# Autodesk Inventor assembly: Assembly
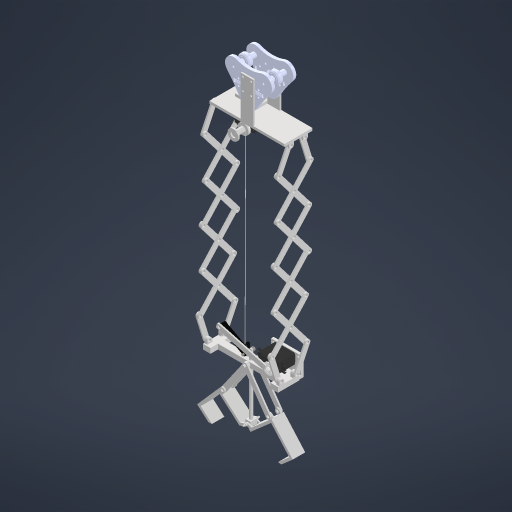
[picture p0: Inventor's stored thumbnail of the model, 512x512]
Saved by Autodesk Inventor 2023.6 (Build 276521000, 521)
## iProperties
Created: 2026-03-04
Part Number: Assembly
Document SubType Name: Assembly
Designer: user
Author: user
## Documents named in this file (19)
- D:\FP Revisi\Assembly.iam
- D:\FP Revisi\Claw New.ipt
- D:\FP Revisi\Claw New side.ipt
- D:\FP Revisi\Claw Connector 1.ipt
- D:\FP Revisi\Shaft.ipt
- D:\FP Revisi\Claw Arm.ipt
- D:\FP Revisi\Claw Connector 2.ipt
- C:\Users\user\OneDrive\Documents\FP V2 Batang Penggerak.ipt
- D:\FP Revisi\MG_996R v1.iam
- C:\Users\user\OneDrive\Documents\Inventor\Content Center Files\R2023\en-US\AS 1420\AS 1420 - 1973 - M4 x 20.ipt
- D:\FP Revisi\Lazy Tongs beam Short.ipt
- D:\FP Revisi\Lazy Tongs beam Long.ipt
- C:\Users\user\Downloads\FP_Batch 2\Sub Assembly Slider axis x.iam
- D:\FP Revisi\Mounting atas.ipt
- C:\Users\user\OneDrive\Documents\fp v2 servo Mounting.ipt
- D:\FP Revisi\MG_996R.iam
- D:\FP Revisi\Pulley Mechanism.ipt
- D:\FP Revisi\Hook.ipt
- D:\FP Revisi\Ropes.ipt
## Components (47 placed, 18 different names)
1. Claw New:1 — Mate:1, Mate:2, Mate:7, Mate:8, Mate:9, Mate:10
2. Claw New side:1 — Mate:1, Mate:2, Mate:3, Mate:4, Mate:11, Mate:12, Mate:13, Mate:14
3. Claw Connector 1:1 — Mate:3, Mate:4, Mate:5, Mate:6
4. Shaft:1 — Mate:5, Mate:6, Mate:18, Mate:20, Mate:26, Mate:35, Mate:36
5. Claw Arm:1 — Mate:11, Mate:12, Mate:15, Mate:19
6. Claw Arm:2 — Mate:7, Mate:8, Mate:15, Mate:16
7. Claw Arm:3 — Mate:9, Mate:10, Mate:17
8. Claw Arm:4 — Mate:13, Mate:14, Mate:16, Mate:17
9. Claw Connector 2:1 — Mate:18, Mate:19, Flush:1, Mate:37, Mate:38, Mate:47, Mate:48, Mate:86, Mate:87, Mate:88, Mate:89, Flush:2, Flush:3, Mate:110, Flush:4, Mate:128, Mate:129
10. FP V2 Batang Penggerak:1 — Mate:20, Mate:23, Mate:24, Mate:25, Mate:34
11. MG_996R v1:1 [sub-assembly] — Flush:1, Mate:23, Mate:24, Mate:27, Mate:32, Flush:3, Mate:111, Mate:112, Mate:113, Mate:114, Mate:115
12. FP V2 Batang Penggerak:2 — Mate:25, Mate:26, Mate:27, Mate:30, Mate:31, Mate:33
13. FP V2 Batang Penggerak:3 — Mate:28, Mate:29, Mate:31, Mate:33
14. FP V2 Batang Penggerak:4 — Mate:28, Mate:29, Mate:30, Mate:32, Mate:34
15. AS 1420 - Metric M4 x 20:1 — Mate:35, Mate:36
16. Lazy Tongs beam Short:4 — Mate:37, Mate:38, Mate:45, Mate:46
17. Lazy Tongs beam Long:1 — Mate:45, Mate:46, Mate:51, Mate:52, Mate:58
18. Lazy Tongs beam Long:2 — Mate:49, Mate:50, Mate:51, Mate:54, Mate:55
19. Lazy Tongs beam Long:3 — Mate:60, Mate:61, Mate:62, Mate:63, Mate:66
20. Lazy Tongs beam Long:4 — Mate:63, Mate:66, Mate:91, Mate:96, Mate:97
21. Lazy Tongs beam Long:5 — Mate:57, Mate:59, Mate:62, Mate:64, Mate:65
22. Lazy Tongs beam Long:6 — Mate:52, Mate:56, Mate:57, Mate:58, Mate:59
23. Lazy Tongs beam Long:7 — Mate:64, Mate:65, Mate:91, Mate:94, Mate:95
24. Lazy Tongs beam Long:8 — Mate:54, Mate:55, Mate:56, Mate:60, Mate:61
25. Lazy Tongs beam Short:5 — Mate:47, Mate:48, Mate:49, Mate:50
26. Lazy Tongs beam Short:6 — Mate:86, Mate:89
27. Lazy Tongs beam Long:9
28. Lazy Tongs beam Long:10
29. Lazy Tongs beam Long:11
30. Lazy Tongs beam Long:12 — Mate:90, Mate:100, Mate:103
31. Lazy Tongs beam Long:13
32. Lazy Tongs beam Long:14
33. Lazy Tongs beam Long:15 — Mate:90, Mate:101, Mate:102
34. Lazy Tongs beam Long:16
35. Lazy Tongs beam Short:7 — Mate:87, Mate:88
36. Mounting atas:1 — Flush:2, Mate:92, Mate:93, Mate:98, Mate:99, Mate:105, Mate:106, Mate:107, Mate:108, Mate:109, Mate:117, Mate:130
37. Lazy Tongs beam Short:9 — Mate:92, Mate:94, Mate:95
38. Lazy Tongs beam Short:10 — Mate:93, Mate:96, Mate:97
39. Lazy Tongs beam Short:11 — Mate:99, Mate:100, Mate:103
40. Lazy Tongs beam Short:12 — Mate:98, Mate:101, Mate:102
41. Sub Assembly Slider axis x:1 [sub-assembly] — Mate:105, Mate:106, Mate:107, Mate:108, Mate:109
42. fp v2 servo Mounting:1 — Mate:110, Mate:111, Mate:112, Mate:113, Mate:114, Mate:115
43. MG_996R:1 [sub-assembly] — Mate:118, Mate:119, Mate:120, Mate:121, Mate:122, Mate:123, Mate:124, Mate:125, Mate:126, Mate:127
44. fp v2 servo Mounting:2 — Mate:117, Mate:118, Mate:119, Mate:120, Mate:121, Mate:122, Mate:130
45. Pulley Mechanism:1 — Mate:123, Mate:124, Mate:125, Mate:126, Mate:127, Flush:4, Flush:5
46. Hook:1 — Mate:128, Mate:129, Flush:6, Flush:9
47. Ropes:1 — Flush:7, Flush:8, Flush:9
## Relationships (128: Mate 119, Flush 9)
- Mate:1: Claw New:1 ↔ Claw New side:1
- Mate:2: Claw New:1 ↔ Claw New side:1
- Mate:3: Claw New side:1 ↔ Claw Connector 1:1
- Mate:4: Claw New side:1 ↔ Claw Connector 1:1
- Mate:5: Claw Connector 1:1 ↔ Shaft:1
- Mate:6: Claw Connector 1:1 ↔ Shaft:1
- Mate:7: Claw New:1 ↔ Claw Arm:2
- Mate:8: Claw New:1 ↔ Claw Arm:2
- Mate:9: Claw New:1 ↔ Claw Arm:3
- Mate:10: Claw New:1 ↔ Claw Arm:3
- Mate:11: Claw New side:1 ↔ Claw Arm:1
- Mate:12: Claw New side:1 ↔ Claw Arm:1
- Mate:13: Claw New side:1 ↔ Claw Arm:4
- Mate:14: Claw New side:1 ↔ Claw Arm:4
- Mate:15: Claw Arm:1 ↔ Claw Arm:2
- Mate:16: Claw Arm:2 ↔ Claw Arm:4
- Mate:17: Claw Arm:3 ↔ Claw Arm:4
- Mate:18: Shaft:1 ↔ Claw Connector 2:1
- Mate:19: Claw Arm:1 ↔ Claw Connector 2:1
- Mate:20: Shaft:1 ↔ FP V2 Batang Penggerak:1
- Flush:1: Claw Connector 2:1 ↔ MG_996R v1:1
- Mate:23: FP V2 Batang Penggerak:1 ↔ MG_996R v1:1
- Mate:24: FP V2 Batang Penggerak:1 ↔ MG_996R v1:1
- Mate:25: FP V2 Batang Penggerak:1 ↔ FP V2 Batang Penggerak:2
- Mate:26: Shaft:1 ↔ FP V2 Batang Penggerak:2
- Mate:27: MG_996R v1:1 ↔ FP V2 Batang Penggerak:2
- Mate:28: FP V2 Batang Penggerak:3 ↔ FP V2 Batang Penggerak:4
- Mate:29: FP V2 Batang Penggerak:3 ↔ FP V2 Batang Penggerak:4
- Mate:30: FP V2 Batang Penggerak:2 ↔ FP V2 Batang Penggerak:4
- Mate:31: FP V2 Batang Penggerak:2 ↔ FP V2 Batang Penggerak:3
- Mate:32: MG_996R v1:1 ↔ FP V2 Batang Penggerak:4
- Mate:33: FP V2 Batang Penggerak:2 ↔ FP V2 Batang Penggerak:3
- Mate:34: FP V2 Batang Penggerak:1 ↔ FP V2 Batang Penggerak:4
- Mate:35: Shaft:1 ↔ AS 1420 - Metric M4 x 20:1
- Mate:36: Shaft:1 ↔ AS 1420 - Metric M4 x 20:1
- Mate:37: Claw Connector 2:1 ↔ Lazy Tongs beam Short:4
- Mate:38: Claw Connector 2:1 ↔ Lazy Tongs beam Short:4
- Mate:45: Lazy Tongs beam Short:4 ↔ Lazy Tongs beam Long:1
- Mate:46: Lazy Tongs beam Short:4 ↔ Lazy Tongs beam Long:1
- Mate:47: Claw Connector 2:1 ↔ Lazy Tongs beam Short:5
- Mate:48: Claw Connector 2:1 ↔ Lazy Tongs beam Short:5
- Mate:49: Lazy Tongs beam Long:2 ↔ Lazy Tongs beam Short:5
- Mate:50: Lazy Tongs beam Long:2 ↔ Lazy Tongs beam Short:5
- Mate:51: Lazy Tongs beam Long:1 ↔ Lazy Tongs beam Long:2
- Mate:52: Lazy Tongs beam Long:1 ↔ Lazy Tongs beam Long:6
- Mate:54: Lazy Tongs beam Long:2 ↔ Lazy Tongs beam Long:8
- Mate:55: Lazy Tongs beam Long:2 ↔ Lazy Tongs beam Long:8
- Mate:56: Lazy Tongs beam Long:6 ↔ Lazy Tongs beam Long:8
- Mate:57: Lazy Tongs beam Long:5 ↔ Lazy Tongs beam Long:6
- Mate:58: Lazy Tongs beam Long:1 ↔ Lazy Tongs beam Long:6
- Mate:59: Lazy Tongs beam Long:5 ↔ Lazy Tongs beam Long:6
- Mate:60: Lazy Tongs beam Long:3 ↔ Lazy Tongs beam Long:8
- Mate:61: Lazy Tongs beam Long:3 ↔ Lazy Tongs beam Long:8
- Mate:62: Lazy Tongs beam Long:3 ↔ Lazy Tongs beam Long:5
- Mate:63: Lazy Tongs beam Long:3 ↔ Lazy Tongs beam Long:4
- Mate:64: Lazy Tongs beam Long:5 ↔ Lazy Tongs beam Long:7
- Mate:65: Lazy Tongs beam Long:5 ↔ Lazy Tongs beam Long:7
- Mate:66: Lazy Tongs beam Long:3 ↔ Lazy Tongs beam Long:4
- [Mate]: Lazy Tongs beam Short:6 ↔ Lazy Tongs beam Long:9
- [Mate]: Lazy Tongs beam Short:6 ↔ Lazy Tongs beam Long:9
- [Mate]: Lazy Tongs beam Long:10 ↔ Lazy Tongs beam Short:7
- [Mate]: Lazy Tongs beam Long:10 ↔ Lazy Tongs beam Short:7
- [Mate]: Lazy Tongs beam Long:9 ↔ Lazy Tongs beam Long:10
- [Mate]: Lazy Tongs beam Long:9 ↔ Lazy Tongs beam Long:14
- [Mate]: Lazy Tongs beam Long:10 ↔ Lazy Tongs beam Long:16
- [Mate]: Lazy Tongs beam Long:10 ↔ Lazy Tongs beam Long:16
- [Mate]: Lazy Tongs beam Long:14 ↔ Lazy Tongs beam Long:16
- [Mate]: Lazy Tongs beam Long:13 ↔ Lazy Tongs beam Long:14
- [Mate]: Lazy Tongs beam Long:9 ↔ Lazy Tongs beam Long:14
- [Mate]: Lazy Tongs beam Long:13 ↔ Lazy Tongs beam Long:14
- [Mate]: Lazy Tongs beam Long:11 ↔ Lazy Tongs beam Long:16
- [Mate]: Lazy Tongs beam Long:11 ↔ Lazy Tongs beam Long:16
- [Mate]: Lazy Tongs beam Long:11 ↔ Lazy Tongs beam Long:13
- [Mate]: Lazy Tongs beam Long:11 ↔ Lazy Tongs beam Long:12
- [Mate]: Lazy Tongs beam Long:13 ↔ Lazy Tongs beam Long:15
- [Mate]: Lazy Tongs beam Long:13 ↔ Lazy Tongs beam Long:15
- [Mate]: Lazy Tongs beam Long:11 ↔ Lazy Tongs beam Long:12
- Mate:86: Claw Connector 2:1 ↔ Lazy Tongs beam Short:6
- Mate:87: Claw Connector 2:1 ↔ Lazy Tongs beam Short:7
- Mate:88: Claw Connector 2:1 ↔ Lazy Tongs beam Short:7
- Mate:89: Claw Connector 2:1 ↔ Lazy Tongs beam Short:6
- Mate:90: Lazy Tongs beam Long:12 ↔ Lazy Tongs beam Long:15
- Mate:91: Lazy Tongs beam Long:4 ↔ Lazy Tongs beam Long:7
- Flush:2: Claw Connector 2:1 ↔ Mounting atas:1
- Mate:92: Mounting atas:1 ↔ Lazy Tongs beam Short:9
- Mate:93: Mounting atas:1 ↔ Lazy Tongs beam Short:10
- Mate:94: Lazy Tongs beam Long:7 ↔ Lazy Tongs beam Short:9
- Mate:95: Lazy Tongs beam Long:7 ↔ Lazy Tongs beam Short:9
- Mate:96: Lazy Tongs beam Long:4 ↔ Lazy Tongs beam Short:10
- Mate:97: Lazy Tongs beam Long:4 ↔ Lazy Tongs beam Short:10
- Mate:98: Mounting atas:1 ↔ Lazy Tongs beam Short:12
- Mate:99: Mounting atas:1 ↔ Lazy Tongs beam Short:11
- Mate:100: Lazy Tongs beam Long:12 ↔ Lazy Tongs beam Short:11
- Mate:101: Lazy Tongs beam Long:15 ↔ Lazy Tongs beam Short:12
- Mate:102: Lazy Tongs beam Long:15 ↔ Lazy Tongs beam Short:12
- Mate:103: Lazy Tongs beam Long:12 ↔ Lazy Tongs beam Short:11
- Mate:105: Mounting atas:1 ↔ Sub Assembly Slider axis x:1
- Mate:106: Mounting atas:1 ↔ Sub Assembly Slider axis x:1
- Mate:107: Mounting atas:1 ↔ Sub Assembly Slider axis x:1
- Mate:108: Mounting atas:1 ↔ Sub Assembly Slider axis x:1
- Mate:109: Mounting atas:1 ↔ Sub Assembly Slider axis x:1
- Flush:3 (16.5 mm): Claw Connector 2:1 ↔ MG_996R v1:1
- Mate:110: Claw Connector 2:1 ↔ fp v2 servo Mounting:1
- Mate:111: MG_996R v1:1 ↔ fp v2 servo Mounting:1
- Mate:112: MG_996R v1:1 ↔ fp v2 servo Mounting:1
- Mate:113: MG_996R v1:1 ↔ fp v2 servo Mounting:1
- Mate:114: MG_996R v1:1 ↔ fp v2 servo Mounting:1
- Mate:115: MG_996R v1:1 ↔ fp v2 servo Mounting:1
- Mate:117: Mounting atas:1 ↔ fp v2 servo Mounting:2
- Mate:118: MG_996R:1 ↔ fp v2 servo Mounting:2
- Mate:119: MG_996R:1 ↔ fp v2 servo Mounting:2
- Mate:120: MG_996R:1 ↔ fp v2 servo Mounting:2
- Mate:121: MG_996R:1 ↔ fp v2 servo Mounting:2
- Mate:122: MG_996R:1 ↔ fp v2 servo Mounting:2
- Mate:123: MG_996R:1 ↔ Pulley Mechanism:1
- Mate:124: MG_996R:1 ↔ Pulley Mechanism:1
- Mate:125: MG_996R:1 ↔ Pulley Mechanism:1
- Mate:126: MG_996R:1 ↔ Pulley Mechanism:1
- Mate:127: MG_996R:1 ↔ Pulley Mechanism:1
- Flush:4: Claw Connector 2:1 ↔ Pulley Mechanism:1
- Mate:128: Claw Connector 2:1 ↔ Hook:1
- Mate:129: Claw Connector 2:1 ↔ Hook:1
- Mate:130: Mounting atas:1 ↔ fp v2 servo Mounting:2
- Flush:5 (1 mm): Pulley Mechanism:1
- Flush:6: Hook:1
- Flush:7: Ropes:1
- Flush:8: Ropes:1
- Flush:9: Hook:1 ↔ Ropes:1
## Named parameters: d121_d49 = 0 mm, d122_d108 = 0 mm, d123_d109 = 0 mm, d124_d110 = 0 mm, d125_d111 = 0 mm, d126_d112 = 0 mm, d127_d113 = 0 mm, d128_d114 = 0 mm, d129_d115 = 0 mm, d130_d116 = 0 mm, d131_d117 = 0 mm, d132_d118 = 0 mm, d133_d119 = 0 mm, d134_d120 = 0 mm, d135_d100 = 0 mm, d136_d103 = 0 mm, d137_d104 = 0 mm, d138_d105 = 0 mm, d139_d106 = 0 mm
